# Autodesk Inventor assembly: Arm V2
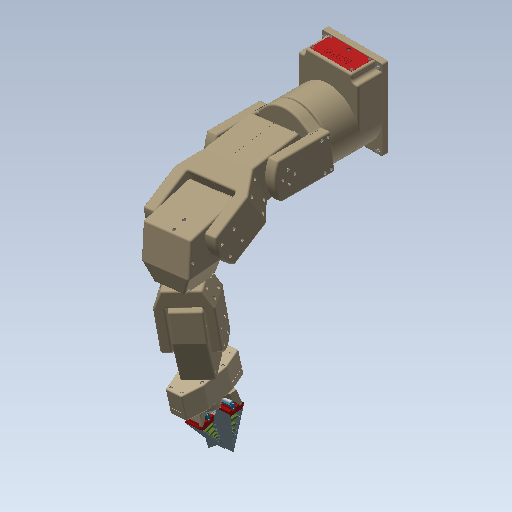
[picture p0: Inventor's stored thumbnail of the model, 512x512]
Saved by Autodesk Inventor 2021 (Build 250183000, 183)
## iProperties
Created: 2020-02-08
Part Number: Arm V2
Document SubType Name: Assembly
Designer: JochenAlt
Author: JochenAlt
## Documents named in this file (8)
- C:\Users\Jochen Alt\Documents\Daten\Projects\MiniBot\CAD\Arm V2.iam
- C:\Users\Jochen Alt\Documents\Daten\Projects\MiniBot\CAD\Elbow V2.iam
- C:\Users\Jochen Alt\Documents\Daten\Projects\MiniBot\CAD\Upperarm.iam
- C:\Users\Jochen Alt\Documents\Daten\Projects\MiniBot\CAD\Base.iam
- C:\Users\Jochen Alt\Documents\Daten\Projects\MiniBot\CAD\Forearm.iam
- C:\Users\Jochen Alt\Documents\Daten\Projects\MiniBot\CAD\Shoulder.iam
- C:\Users\Jochen Alt\Documents\Daten\Projects\MiniBot\CAD\Wrist.iam
- C:\Users\Jochen Alt\Documents\Daten\Projects\MiniBot\CAD\gripper\Gripper.iam
## Components (7 placed, 7 different names)
1. Upperarm:1 [sub-assembly] — Passend:69, Passend:70, Passend:82, Passend:83
2. Base:1 [sub-assembly] — Passend:61, Fluchtend:1
3. Shoulder:1 [sub-assembly] — Passend:61, Fluchtend:1, Passend:82, Passend:83
4. Elbow:2 [sub-assembly] — Passend:69, Passend:70, Passend:77, Passend:78
5. Wrist:3 [sub-assembly] — Passend:75, Passend:79, Passend:80, Passend:81, Passend:84, Mate:85
6. Gripper:1 [sub-assembly] — Passend:75, Passend:81, Passend:84, Mate:85
7. Forearm:1 [sub-assembly] — Passend:77, Passend:78, Passend:79, Passend:80
## Relationships (14: Mate 13, Flush 1)
- Passend:61 [Mate]: Base:1 ↔ Shoulder:1
- Fluchtend:1 [Flush]: Base:1 ↔ Shoulder:1
- Passend:69 [Mate]: Upperarm:1 ↔ Elbow:2
- Passend:70 [Mate]: Upperarm:1 ↔ Elbow:2
- Passend:75 [Mate]: Wrist:3 ↔ Gripper:1
- Passend:77 [Mate]: Elbow:2 ↔ Forearm:1
- Passend:78 [Mate]: Elbow:2 ↔ Forearm:1
- Passend:79 [Mate]: Wrist:3 ↔ Forearm:1
- Passend:80 [Mate]: Wrist:3 ↔ Forearm:1
- Passend:81 [Mate]: Wrist:3 ↔ Gripper:1
- Passend:82 [Mate]: Upperarm:1 ↔ Shoulder:1
- Passend:83 [Mate]: Upperarm:1 ↔ Shoulder:1
- Passend:84 [Mate]: Wrist:3 ↔ Gripper:1
- Mate:85 (1 mm): Wrist:3 ↔ Gripper:1
